# Autodesk Inventor assembly: obudowa - czujnik czadu
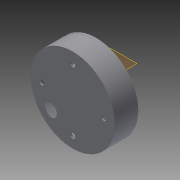
[picture p0: Inventor's stored thumbnail of the model, 180x180]
Saved by Autodesk Inventor 2014 (Build 180170000, 170)
## iProperties
Created: 2018-02-27
Part Number: obudowa - czujnik czadu
Document SubType Name: Assembly
Designer: HP820
Author: HP820
## Documents named in this file (3)
- C:\Users\HP820\Dysk Google\Projekt SYSTEM POWIADOMIEN DLA OSOB GLUCHONIEMYCH I NIEDOSLYSZACYCH BY JACEK MARTYNIAK I ŁUKASZ NOWARKIEWICZ\Projekty 3D obudowy\obudowa - czujnik czadu\obudowa - czujnik czadu.iam
- C:\Users\HP820\Dysk Google\Projekt SYSTEM POWIADOMIEN DLA OSOB GLUCHONIEMYCH I NIEDOSLYSZACYCH BY JACEK MARTYNIAK I ŁUKASZ NOWARKIEWICZ\Projekty 3D obudowy\obudowa - czujnik czadu\obudowa - czujnik czadu - dol.ipt
- C:\Users\HP820\Dysk Google\Projekt SYSTEM POWIADOMIEN DLA OSOB GLUCHONIEMYCH I NIEDOSLYSZACYCH BY JACEK MARTYNIAK I ŁUKASZ NOWARKIEWICZ\Projekty 3D obudowy\obudowa - czujnik czadu\obudowa - czujnik czadu - gora.ipt
## Components (2 placed, 2 different names)
1. obudowa - czujnik czadu - dol:1 — Flush:1
2. obudowa - czujnik czadu - gora:1 — Flush:1
## Relationships (1: Flush 1)
- Flush:1: obudowa - czujnik czadu - dol:1 ↔ obudowa - czujnik czadu - gora:1
